# Autodesk Inventor assembly: microvendoor
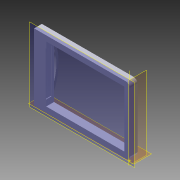
[picture p0: Inventor's stored thumbnail of the model, 180x180]
Saved by Autodesk Inventor 2015 (Build 190159000, 159)
## iProperties
Created: 2015-10-18
Part Number: microvendoor
Document SubType Name: Assembly
Designer: omae
Author: omae
## Documents named in this file (2)
- C:\Users\omae\Desktop\研究室\論文・資料\ROS\kitchen\stl\microvendoor.iam
- C:\Users\omae\Desktop\研究室\論文・資料\ROS\kitchen\toolinstall\homeIsland\summerSeminar\micorooven\microwaveOvenDoor.ipt
## Components (1 placed, 1 different names)
1. microwaveOvenDoor:1 — メイト:1, メイト:2, フラッシュ:1
## Relationships (3: Mate 2, Flush 1)
- メイト:1 [Mate]: microwaveOvenDoor:1
- メイト:2 [Mate]: microwaveOvenDoor:1
- フラッシュ:1 [Flush]: microwaveOvenDoor:1
